# Autodesk Inventor assembly: RearmostAftSectionAssembly0
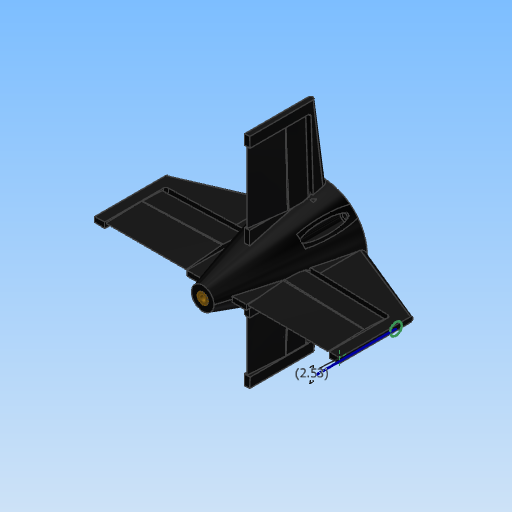
[picture p0: Inventor's stored thumbnail of the model, 512x512]
Saved by Autodesk Inventor 2017 (Build 210142000, 142)
## iProperties
Created: 2016-10-06
Part Number: RearmostAftSectionAssembly0
Document SubType Name: Assembly
Designer: techn
Author: techn
## Documents named in this file (14)
- D:\OneDrive\Documents\Other Projects\Submarine\CAD\aft\RearmostAftSectionAssembly0.iam
- D:\OneDrive\Documents\Other Projects\Submarine\CAD\aft\RearmostAftSection.ipt
- D:\OneDrive\Documents\Other Projects\Submarine\CAD\aft\SleeveBearing4mmFlanged.ipt
- D:\OneDrive\Documents\Other Projects\Submarine\CAD\common\SleeveBearing3mmFlanged.ipt
- D:\OneDrive\Documents\Other Projects\Submarine\CAD\common\steeringYoke3mmShaft.ipt
- D:\OneDrive\Documents\Other Projects\Submarine\CAD\aft\RudderStabilizingFins.ipt
- D:\OneDrive\Documents\Other Projects\Submarine\CAD\aft\RudderStabilizingFinBottom.ipt
- D:\OneDrive\Documents\Other Projects\Submarine\CAD\aft\RudderStabilizingLowerFins.ipt
- D:\OneDrive\Documents\Other Projects\Submarine\CAD\aft\DivePlanesStabilizingFins.ipt
- D:\OneDrive\Documents\Other Projects\Submarine\CAD\aft\RudderUpperControlSurface.ipt
- D:\OneDrive\Documents\Other Projects\Submarine\CAD\aft\RudderLowerControlSurface.ipt
- D:\OneDrive\Documents\Other Projects\Submarine\CAD\aft\DivePlanesControlSurface.ipt
- D:\OneDrive\Documents\Other Projects\Submarine\CAD\aft\3mmControlSurfaceShaft_1.ipt
- D:\OneDrive\Documents\Other Projects\Submarine\CAD\aft\3mmControlSurfaceShaft_2.ipt
## Components (24 placed, 13 different names)
1. RearmostAftSection:1 — Mate:1, Mate:2, Mate:3, Mate:4, Mate:5, Mate:8, Mate:9, Mate:10, Mate:11, Mate:14, Mate:15, Mate:16, Angle:1, Mate:17, Mate:18, Angle:2, Mate:19, Mate:20, Mate:21, Mate:22, Mate:23, Mate:24, Mate:25, Mate:26, Angle:3, Mate:27, Mate:28, Angle:4, Mate:29, Mate:30, Mate:31, Mate:32, Mate:33, Mate:34
2. SleeveBearing4mmFlanged:1 — Mate:1, Mate:14
3. SleeveBearing3mmFlanged:1 — Mate:2, Mate:7, Mate:8, Mate:12, Mate:35, Mate:36, Mate:53
4. steeringYoke3mmShaft:1 — Mate:7, Mate:12
5. steeringYoke3mmShaft:2 — Mate:6, Mate:13
6. SleeveBearing3mmFlanged:2 — Mate:4, Mate:6, Mate:9, Mate:41, Mate:42, Mate:45
7. SleeveBearing3mmFlanged:3 — Mate:3, Mate:10, Mate:13, Mate:39, Mate:40, Mate:51
8. SleeveBearing3mmFlanged:4 — Mate:5, Mate:11, Mate:37, Mate:38, Mate:55
9. RudderStabilizingFins:1 — Mate:15, Mate:16, Angle:1
10. RudderStabilizingFinBottom:1 — Mate:17, Mate:18, Angle:2
11. RudderStabilizingLowerFins:1 — Mate:21, Mate:22, Mate:23
12. RudderStabilizingLowerFins:2 — Mate:19, Mate:20, Mate:24
13. DivePlanesStabilizingFins:1 — Mate:25, Mate:26, Angle:3
14. DivePlanesStabilizingFins:2 — Mate:27, Mate:28, Angle:4
15. RudderStabilizingLowerFins:3 — Mate:29, Mate:30, Mate:31
16. RudderStabilizingLowerFins:4 — Mate:32, Mate:33, Mate:34
17. RudderUpperControlSurface:1 — Mate:35, Mate:36, Mate:44, Mate:54
18. RudderLowerControlSurface:1 — Mate:37, Mate:38, Mate:44, Mate:56
19. DivePlanesControlSurface:1 — Mate:41, Mate:42, Mate:43, Mate:46
20. DivePlanesControlSurface:2 — Mate:39, Mate:40, Mate:43, Mate:52
21. 3mmControlSurfaceShaft_1:1 — Mate:45, Mate:46
22. 3mmControlSurfaceShaft_1:3 — Mate:51, Mate:52
23. 3mmControlSurfaceShaft_2:1 — Mate:55, Mate:56
24. 3mmControlSurfaceShaft_2:2 — Mate:53, Mate:54
## Relationships (56: Mate 52, Angle 4)
- Mate:1: RearmostAftSection:1 ↔ SleeveBearing4mmFlanged:1
- Mate:2: RearmostAftSection:1 ↔ SleeveBearing3mmFlanged:1
- Mate:3: RearmostAftSection:1 ↔ SleeveBearing3mmFlanged:3
- Mate:4: RearmostAftSection:1 ↔ SleeveBearing3mmFlanged:2
- Mate:5: RearmostAftSection:1 ↔ SleeveBearing3mmFlanged:4
- Mate:6: steeringYoke3mmShaft:2 ↔ SleeveBearing3mmFlanged:2
- Mate:7: SleeveBearing3mmFlanged:1 ↔ steeringYoke3mmShaft:1
- Mate:8: RearmostAftSection:1 ↔ SleeveBearing3mmFlanged:1
- Mate:9: RearmostAftSection:1 ↔ SleeveBearing3mmFlanged:2
- Mate:10: RearmostAftSection:1 ↔ SleeveBearing3mmFlanged:3
- Mate:11: RearmostAftSection:1 ↔ SleeveBearing3mmFlanged:4
- Mate:12 (6.2433 mm): SleeveBearing3mmFlanged:1 ↔ steeringYoke3mmShaft:1
- Mate:13 (1.3538 mm): steeringYoke3mmShaft:2 ↔ SleeveBearing3mmFlanged:3
- Mate:14: RearmostAftSection:1 ↔ SleeveBearing4mmFlanged:1
- Mate:15: RearmostAftSection:1 ↔ RudderStabilizingFins:1
- Mate:16: RearmostAftSection:1 ↔ RudderStabilizingFins:1
- Angle:1 (0 deg): RearmostAftSection:1 ↔ RudderStabilizingFins:1
- Mate:17: RearmostAftSection:1 ↔ RudderStabilizingFinBottom:1
- Mate:18: RearmostAftSection:1 ↔ RudderStabilizingFinBottom:1
- Angle:2 (0 deg): RearmostAftSection:1 ↔ RudderStabilizingFinBottom:1
- Mate:19: RearmostAftSection:1 ↔ RudderStabilizingLowerFins:2
- Mate:20: RearmostAftSection:1 ↔ RudderStabilizingLowerFins:2
- Mate:21: RearmostAftSection:1 ↔ RudderStabilizingLowerFins:1
- Mate:22: RearmostAftSection:1 ↔ RudderStabilizingLowerFins:1
- Mate:23: RearmostAftSection:1 ↔ RudderStabilizingLowerFins:1
- Mate:24: RearmostAftSection:1 ↔ RudderStabilizingLowerFins:2
- Mate:25: RearmostAftSection:1 ↔ DivePlanesStabilizingFins:1
- Mate:26: RearmostAftSection:1 ↔ DivePlanesStabilizingFins:1
- Angle:3 (0 deg): RearmostAftSection:1 ↔ DivePlanesStabilizingFins:1
- Mate:27: RearmostAftSection:1 ↔ DivePlanesStabilizingFins:2
- Mate:28: RearmostAftSection:1 ↔ DivePlanesStabilizingFins:2
- Angle:4 (0 deg): RearmostAftSection:1 ↔ DivePlanesStabilizingFins:2
- Mate:29: RearmostAftSection:1 ↔ RudderStabilizingLowerFins:3
- Mate:30: RearmostAftSection:1 ↔ RudderStabilizingLowerFins:3
- Mate:31: RearmostAftSection:1 ↔ RudderStabilizingLowerFins:3
- Mate:32: RearmostAftSection:1 ↔ RudderStabilizingLowerFins:4
- Mate:33: RearmostAftSection:1 ↔ RudderStabilizingLowerFins:4
- Mate:34: RearmostAftSection:1 ↔ RudderStabilizingLowerFins:4
- Mate:35: SleeveBearing3mmFlanged:1 ↔ RudderUpperControlSurface:1
- Mate:36 (1.5875 mm): SleeveBearing3mmFlanged:1 ↔ RudderUpperControlSurface:1
- Mate:37: SleeveBearing3mmFlanged:4 ↔ RudderLowerControlSurface:1
- Mate:38 (1.5875 mm): SleeveBearing3mmFlanged:4 ↔ RudderLowerControlSurface:1
- Mate:39: SleeveBearing3mmFlanged:3 ↔ DivePlanesControlSurface:2
- Mate:40 (1.5875 mm): SleeveBearing3mmFlanged:3 ↔ DivePlanesControlSurface:2
- Mate:41: SleeveBearing3mmFlanged:2 ↔ DivePlanesControlSurface:1
- Mate:42 (1.5875 mm): SleeveBearing3mmFlanged:2 ↔ DivePlanesControlSurface:1
- Mate:43: DivePlanesControlSurface:1 ↔ DivePlanesControlSurface:2
- Mate:44: RudderUpperControlSurface:1 ↔ RudderLowerControlSurface:1
- Mate:45: SleeveBearing3mmFlanged:2 ↔ 3mmControlSurfaceShaft_1:1
- Mate:46: DivePlanesControlSurface:1 ↔ 3mmControlSurfaceShaft_1:1
- Mate:51: SleeveBearing3mmFlanged:3 ↔ 3mmControlSurfaceShaft_1:3
- Mate:52: DivePlanesControlSurface:2 ↔ 3mmControlSurfaceShaft_1:3
- Mate:53: SleeveBearing3mmFlanged:1 ↔ 3mmControlSurfaceShaft_2:2
- Mate:54: RudderUpperControlSurface:1 ↔ 3mmControlSurfaceShaft_2:2
- Mate:55: SleeveBearing3mmFlanged:4 ↔ 3mmControlSurfaceShaft_2:1
- Mate:56: RudderLowerControlSurface:1 ↔ 3mmControlSurfaceShaft_2:1
